# Autodesk Inventor assembly: Собранная Мясорубка
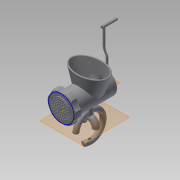
[picture p0: Inventor's stored thumbnail of the model, 180x180]
Saved by Autodesk Inventor 2014 SP1 (Build 180222100, 222)
## iProperties
Created: 2023-07-20
Part Number: Собранная Мясорубка
Document SubType Name: Assembly
Designer: 1.507-10
Author: 1.507-10
## Documents named in this file (7)
- C:\Users\1.507-10\Documents\Inventor\kirogagl\Собранная Мясорубка.iam
- C:\Users\1.507-10\Documents\Inventor\kirogagl\Крышка.ipt
- C:\Users\1.507-10\Documents\Inventor\kirogagl\Матрица.ipt
- C:\Users\1.507-10\Documents\Inventor\kirogagl\Нож.ipt
- C:\Users\1.507-10\Documents\Inventor\kirogagl\Рукоять.ipt
- C:\Users\1.507-10\Documents\Inventor\kirogagl\Шнек.ipt
- C:\Users\1.507-10\Documents\Inventor\kirogagl\Корпус.ipt
## Components (6 placed, 6 different names)
1. Крышка:1 — Вращательный:2
2. Матрица:1 — Вращательный:2, Жесткий:2
3. Нож:1 — Жесткий:1
4. Рукоять:1 — Вращательный:3
5. Шнек:1 — Жесткий:1, Вращательный:1, Жесткий:2
6. Корпус:1 — Вращательный:1, Вращательный:3
## Relationships (5: RevoluteJoint 3, WeldJoint 2)
- Жесткий:1 [WeldJoint]: Нож:1 ↔ Шнек:1
- Вращательный:1 [RevoluteJoint]: Шнек:1 ↔ Корпус:1
- Вращательный:2 [RevoluteJoint]: Крышка:1 ↔ Матрица:1
- Жесткий:2 [WeldJoint]: Матрица:1 ↔ Шнек:1
- Вращательный:3 [RevoluteJoint]: Рукоять:1 ↔ Корпус:1
